# Autodesk Inventor assembly: Shooter Assembly
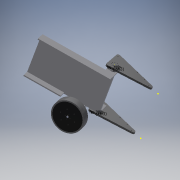
[picture p0: Inventor's stored thumbnail of the model, 180x180]
Saved by Autodesk Inventor 2019 (Build 230136000, 136)
## iProperties
Created: 2020-10-17
Part Number: Shooter Assembly
Document SubType Name: Assembly
Designer: Delta
Author: Delta
## Documents named in this file (7)
- C:\Robotics\2020-21-CAD\Shooter\Shooter Assembly.iam
- C:\Robotics\2020-21-CAD\Shooter\Guide.ipt
- C:\Robotics\2020-21-CAD\Shooter\Axle Rotate.ipt
- C:\Robotics\2020-21-CAD\Shooter\Triangle axle slide connector.ipt
- C:\Robotics\2020-21-CAD\Shooter\Tetrex 2pc motor mount.ipt
- C:\Robotics\2020-21-CAD\Shooter\motor-3102NeveRest20 (1).ipt
- C:\Robotics\2020-21-CAD\Shooter\Flywheel_4inWheel8mmHub.ipt
## Components (8 placed, 6 different names)
1. Guide:1 — Mate:1, Mate:2, Mate:3, Mate:4, Mate:5, Mate:6, Mate:14, Mate:15, Angle:1, Angle:2
2. Axle Rotate:1 — Mate:1, Mate:2, Mate:3, Mate:9, Mate:13
3. Axle Rotate:2 — Mate:4, Mate:5, Mate:6, Mate:8, Mate:12
4. Triangle axle slide connector:1 — Mate:8, Flush:2, Mate:12
5. Triangle axle slide connector:2 — Mate:9, Flush:2, Mate:13
6. Tetrex 2pc motor mount:1 — Mate:14, Mate:15, Angle:1, Mate:16, Mate:17
7. motor-3102NeveRest20 (1):1 — Mate:16, Mate:17, Mate:18, Mate:19, Angle:2
8. Flywheel_4inWheel8mmHub:1 — Mate:18, Mate:19
## Relationships (19: Mate 16, Angle 2, Flush 1)
- Mate:1: Guide:1 ↔ Axle Rotate:1
- Mate:2: Guide:1 ↔ Axle Rotate:1
- Mate:3: Guide:1 ↔ Axle Rotate:1
- Mate:4: Guide:1 ↔ Axle Rotate:2
- Mate:5: Guide:1 ↔ Axle Rotate:2
- Mate:6: Guide:1 ↔ Axle Rotate:2
- Mate:8: Axle Rotate:2 ↔ Triangle axle slide connector:1
- Mate:9: Axle Rotate:1 ↔ Triangle axle slide connector:2
- Flush:2: Triangle axle slide connector:1 ↔ Triangle axle slide connector:2
- Mate:12: Axle Rotate:2 ↔ Triangle axle slide connector:1
- Mate:13: Axle Rotate:1 ↔ Triangle axle slide connector:2
- Mate:14: Guide:1 ↔ Tetrex 2pc motor mount:1
- Mate:15: Guide:1 ↔ Tetrex 2pc motor mount:1
- Angle:1 (0 deg): Guide:1 ↔ Tetrex 2pc motor mount:1
- Mate:16: Tetrex 2pc motor mount:1 ↔ motor-3102NeveRest20 (1):1
- Mate:17: Tetrex 2pc motor mount:1 ↔ motor-3102NeveRest20 (1):1
- Mate:18: motor-3102NeveRest20 (1):1 ↔ Flywheel_4inWheel8mmHub:1
- Mate:19: motor-3102NeveRest20 (1):1 ↔ Flywheel_4inWheel8mmHub:1
- Angle:2 (0 deg): Guide:1 ↔ motor-3102NeveRest20 (1):1
